# Autodesk Inventor assembly: E002_Canon
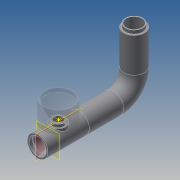
[picture p0: Inventor's stored thumbnail of the model, 180x180]
Saved by Autodesk Inventor 2020 (Build 240168000, 168)
## iProperties
Created: 2021-10-15
Part Number: E002_Canon
Document SubType Name: Assembly
Designer: gabri
Author: gabri
## Documents named in this file (7)
- D:\PGA\E002_Canon.iam
- D:\PGA\P007_CanonSupportRervoir.ipt
- D:\PGA\P006_CanonConfettis.ipt
- D:\PGA\P008_CanonBout.ipt
- D:\PGA\P009_CanonAdaptateurReservoir.ipt
- D:\PGA\P010_CanonCoude.ipt
- D:\PGA\P013_Canon_venturiCoudé.ipt
## Components (7 placed, 6 different names)
1. P007_CanonSupportRervoir:1 — Placage:1, Placage:2, Placage:3, Logement:1, Logement:2, Logement:3
2. P006_CanonConfettis:1 — Logement:1
3. P008_CanonBout:1 — Logement:5
4. P008_CanonBout:2 — Logement:3, Logement:4
5. P009_CanonAdaptateurReservoir:1 — Logement:2, Angle:1, Placage:4
6. P010_CanonCoude:1 — Logement:4, Angle:1, Logement:5
7. P013_Canon_venturiCoudé:1 — Placage:4
## Relationships (10: Insert 5, Mate 4, Angle 1)
- Placage:1 [Mate]: P007_CanonSupportRervoir:1
- Placage:2 [Mate]: P007_CanonSupportRervoir:1
- Placage:3 [Mate]: P007_CanonSupportRervoir:1
- Logement:1 [Insert]: P007_CanonSupportRervoir:1 ↔ P006_CanonConfettis:1
- Logement:2 [Insert]: P007_CanonSupportRervoir:1 ↔ P009_CanonAdaptateurReservoir:1
- Logement:3 [Insert]: P007_CanonSupportRervoir:1 ↔ P008_CanonBout:2
- Logement:4 [Insert]: P008_CanonBout:2 ↔ P010_CanonCoude:1
- Angle:1 (0 deg): P009_CanonAdaptateurReservoir:1 ↔ P010_CanonCoude:1
- Logement:5 [Insert]: P008_CanonBout:1 ↔ P010_CanonCoude:1
- Placage:4 [Mate]: P009_CanonAdaptateurReservoir:1 ↔ P013_Canon_venturiCoudé:1
